# Autodesk Inventor assembly: A2017_T2_04
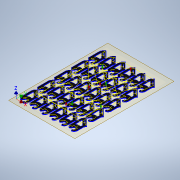
[picture p0: Inventor's stored thumbnail of the model, 180x180]
Saved by Autodesk Inventor 2022 (Build 260153000, 153)
## iProperties
Created: 2022-09-28
Part Number: A2017_T2_04
Document SubType Name: Assembly
Designer: Masato
Author: Masato
## Documents named in this file (3)
- C:\Users\6343y\ドキュメント\Inventor\SUSTAINA-OP\Cam\A2017_T2\A2017_T2_04.iam
- C:\Users\6343y\ドキュメント\Inventor\SUSTAINA-OP\Cam\DisposableBoard.ipt
- C:\Users\6343y\ドキュメント\Inventor\SUSTAINA-OP\UpperBody\Arm\Shoulder_side_frame.ipt
## Components (31 placed, 2 different names)
1. DisposableBoard:1 — フラッシュ:1, フラッシュ:2, フラッシュ:3, フラッシュ:4, フラッシュ:5, 正接:1
2. Shoulder_side_frame:1 — メイト:1, フラッシュ:5, 正接:1
3. Shoulder_side_frame:2
4. Shoulder_side_frame:3
5. Shoulder_side_frame:4
6. Shoulder_side_frame:5
7. Shoulder_side_frame:6
8. Shoulder_side_frame:7
9. Shoulder_side_frame:8
10. Shoulder_side_frame:9
11. Shoulder_side_frame:10
12. Shoulder_side_frame:11
13. Shoulder_side_frame:12
14. Shoulder_side_frame:13
15. Shoulder_side_frame:14
16. Shoulder_side_frame:15
17. Shoulder_side_frame:16
18. Shoulder_side_frame:17
19. Shoulder_side_frame:18
20. Shoulder_side_frame:19
21. Shoulder_side_frame:20
22. Shoulder_side_frame:21
23. Shoulder_side_frame:22
24. Shoulder_side_frame:23
25. Shoulder_side_frame:24
26. Shoulder_side_frame:25
27. Shoulder_side_frame:26
28. Shoulder_side_frame:27
29. Shoulder_side_frame:28
30. Shoulder_side_frame:29
31. Shoulder_side_frame:30
## Component patterns: (30 elements, first: Shoulder_side_frame:1)
## Relationships (7: Flush 5, Mate 1, Tangent 1)
- フラッシュ:1 [Flush]: DisposableBoard:1
- フラッシュ:2 [Flush]: DisposableBoard:1
- フラッシュ:3 [Flush]: DisposableBoard:1
- フラッシュ:4 [Flush]: DisposableBoard:1
- メイト:1 [Mate]: Shoulder_side_frame:1
- フラッシュ:5 [Flush] (2 mm): DisposableBoard:1 ↔ Shoulder_side_frame:1
- 正接:1 [Tangent] (2 mm): DisposableBoard:1 ↔ Shoulder_side_frame:1
